# Autodesk Inventor assembly: LFR
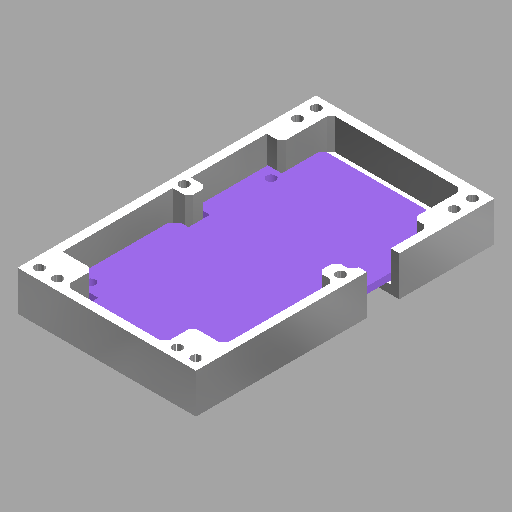
[picture p0: Inventor's stored thumbnail of the model, 512x512]
Saved by Autodesk Inventor 2022 (Build 260153000, 153)
## iProperties
Created: 2021-10-06
Part Number: LFR
Document SubType Name: Assembly
Designer: Bowen O'Steen
Author: Bowen O'Steen
## Documents named in this file (3)
- C:\Users\gwhen\OneDrive\Desktop\Vault\Designs\MEMESat\MemeSat\Engineering Data\MemeSat\Subsystems\LFR\LFR.iam
- C:\Users\gwhen\OneDrive\Desktop\Vault\Designs\MEMESat\MemeSat\Engineering Data\MemeSat\Subsystems\LFR\LFRshroud.ipt
- C:\Users\gwhen\OneDrive\Desktop\Vault\Designs\MEMESat\MemeSat\Engineering Data\MemeSat\Subsystems\LFR\LFRboard.ipt
## Components (2 placed, 2 different names)
1. LFRshroud:1 — Mate:1, Flush:1, Mate:2, Mate:3, Mate:4, Mate:5
2. LFRboard:1 — Mate:3, Mate:4, Mate:5
## Relationships (6: Mate 5, Flush 1)
- Mate:1: LFRshroud:1
- Flush:1: LFRshroud:1
- Mate:2: LFRshroud:1
- Mate:3: LFRshroud:1 ↔ LFRboard:1
- Mate:4: LFRshroud:1 ↔ LFRboard:1
- Mate:5: LFRshroud:1 ↔ LFRboard:1
